# Autodesk Inventor assembly: MainTurretAssembly
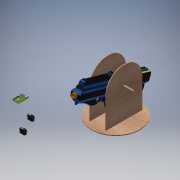
[picture p0: Inventor's stored thumbnail of the model, 180x180]
Saved by Autodesk Inventor 2018 (Build 220112000, 112)
## iProperties
Created: 2019-02-20
Part Number: MainTurretAssembly
Document SubType Name: Assembly
Designer: snipe
Author: snipe
## Documents named in this file (9)
- C:\Users\snipe\Documents\CPRE186-CAD\MainTurretAssembly.iam
- C:\Users\snipe\Documents\CPRE186-CAD\NerfRivalZeus.ipt
- C:\Users\snipe\Documents\CPRE186-CAD\Raspi3B+_Mockup.ipt
- C:\Users\snipe\Documents\CPRE186-CAD\Servo.iam
- C:\Users\snipe\Documents\CPRE186-CAD\turretBasePlate.ipt
- C:\Users\snipe\Documents\CPRE186-CAD\turretSidePlateOne.ipt
- C:\Users\snipe\Documents\CPRE186-CAD\turretSidePlateTwo.ipt
- C:\Users\snipe\Documents\CPRE186-CAD\0.5inHexBearing.ipt
- C:\Users\snipe\Documents\CPRE186-CAD\HexShaft12in.ipt
## Components (10 placed, 8 different names)
1. NerfRivalZeus:1 — Flush:1, Flush:2, Flush:3
2. Raspi3B+_Mockup:1
3. Servo:1 [sub-assembly]
4. Servo:2 [sub-assembly]
5. turretBasePlate:1 — Mate:1, Mate:2, Mate:3, Mate:4, Mate:5, Mate:6
6. turretSidePlateOne:1 — Mate:1, Mate:2, Mate:3, Mate:7, Mate:8, Symmetry:1
7. turretSidePlateTwo:1 — Mate:4, Mate:5, Mate:6, Mate:9, Mate:10, Symmetry:1
8. 0.5inHexBearing:1 — Mate:7, Mate:8, Mate:11, Mate:12
9. 0.5inHexBearing:2 — Mate:9, Mate:10, Mate:13
10. HexShaft12in:1 — Mate:11, Mate:12, Mate:13, Flush:1, Flush:2, Flush:3
## Relationships (17: Mate 13, Flush 3, Symmetry 1)
- Mate:1: turretBasePlate:1 ↔ turretSidePlateOne:1
- Mate:2: turretBasePlate:1 ↔ turretSidePlateOne:1
- Mate:3: turretBasePlate:1 ↔ turretSidePlateOne:1
- Mate:4: turretBasePlate:1 ↔ turretSidePlateTwo:1
- Mate:5: turretBasePlate:1 ↔ turretSidePlateTwo:1
- Mate:6: turretBasePlate:1 ↔ turretSidePlateTwo:1
- Mate:7: turretSidePlateOne:1 ↔ 0.5inHexBearing:1
- Mate:8: turretSidePlateOne:1 ↔ 0.5inHexBearing:1
- Mate:9: turretSidePlateTwo:1 ↔ 0.5inHexBearing:2
- Mate:10: turretSidePlateTwo:1 ↔ 0.5inHexBearing:2
- Mate:11: 0.5inHexBearing:1 ↔ HexShaft12in:1
- Mate:12: 0.5inHexBearing:1 ↔ HexShaft12in:1
- Mate:13: 0.5inHexBearing:2 ↔ HexShaft12in:1
- Flush:1: NerfRivalZeus:1 ↔ HexShaft12in:1
- Flush:2: NerfRivalZeus:1 ↔ HexShaft12in:1
- Flush:3: NerfRivalZeus:1 ↔ HexShaft12in:1
- Symmetry:1: turretSidePlateOne:1 ↔ turretSidePlateTwo:1
